# Autodesk Inventor assembly: ABD_Version 1.0
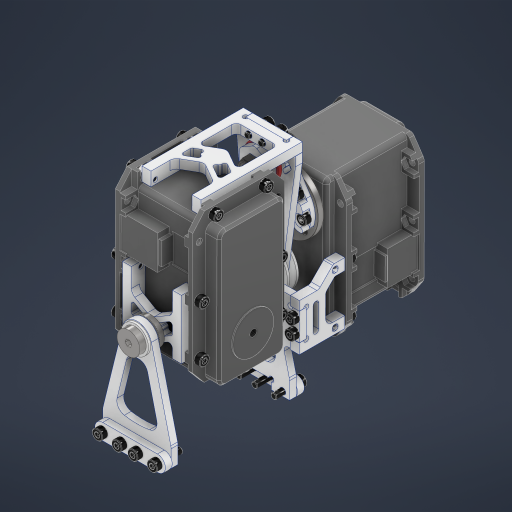
[picture p0: Inventor's stored thumbnail of the model, 512x512]
Saved by Autodesk Inventor 2024 (Build 280153000, 153)
## iProperties
Created: 2024-01-25
Part Number: ABD_Version 1.0
Document SubType Name: Assembly
Designer: ASUS
Author: ASUS
## Documents named in this file (6)
- C:\Users\ASUS\Desktop\Anti_Backlash_Structure_OP\v2_Frame\ABD_V2_Right_OP.iam
- C:\Users\ASUS\Desktop\Anti_Backlash_Structure_OP\MISUMI\Crank_Slider_Fixer.iam
- C:\Users\ASUS\Desktop\Anti_Backlash_Structure_OP\v2_Frame\ABD_MX_64_Roll_Fixation_Set.iam
- C:\Users\ASUS\Desktop\Anti_Backlash_Structure_OP\v2_Frame\ABD_Slider_Set.iam
- C:\Users\ASUS\Desktop\Anti_Backlash_Structure_OP\v2_Frame\Roll_Fixation_Set.iam
- C:\Users\ASUS\Desktop\Anti_Backlash_Structure_OP\v2_Frame\ABD_MX_64_Slider_Fixation_Set_Left2Horn.iam
## Components (5 placed, 5 different names)
1. ABD_MX_64_Roll_Fixation_Set:1 [sub-assembly]
2. ABD_Slider_Set:1 [sub-assembly]
3. Roll_Fixation_Set:1 [sub-assembly]
4. Crank_Slider_Fixer:1 [sub-assembly]
5. ABD_MX_64_Slider_Fixation_Set_Left2Horn:1 [sub-assembly]
## Relationships (7: Mate 4, Insert 3)
- [Insert]: ABD_Slider_Set:1 ↔ Roll_Fixation_Set:1
- [Insert]: ABD_MX_64_Roll_Fixation_Set:1 ↔ Roll_Fixation_Set:1
- [Insert]: ABD_Slider_Set:1 ↔ Crank_Slider_Fixer:1
- [Mate] (0.025 mm): Crank_Slider_Fixer:1 ↔ ABD_MX_64_Slider_Fixation_Set_Left2Horn:1
- [Mate]: ABD_MX_64_Roll_Fixation_Set:1 ↔ ABD_MX_64_Slider_Fixation_Set_Left2Horn:1
- [Mate]: ABD_MX_64_Roll_Fixation_Set:1 ↔ ABD_MX_64_Slider_Fixation_Set_Left2Horn:1
- [Mate] (0.05 mm): ABD_MX_64_Roll_Fixation_Set:1 ↔ ABD_MX_64_Slider_Fixation_Set_Left2Horn:1
## Named parameters: d191_d198 = 0 mm, d192_d199 = 0 mm, d193_d200 = 0.05 mm
